# Autodesk Inventor assembly: манипулятор3
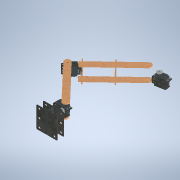
[picture p0: Inventor's stored thumbnail of the model, 180x180]
Saved by Autodesk Inventor 2020.1 (Build 241239000, 239)
## iProperties
Created: 2021-08-18
Part Number: манипулятор3
Document SubType Name: Assembly
Designer: User
Author: User
## Documents named in this file (8)
- D:\GitHub\avatar-kvantoriada\3D\манипулятор3.iam
- D:\GitHub\avatar-kvantoriada\3D\основа.ipt
- D:\GitHub\avatar-kvantoriada\3D\сборка серва 90.iam
- D:\GitHub\avatar-kvantoriada\3D\сборка серва 45_ЗЕРКАЛО2.iam
- D:\GitHub\avatar-kvantoriada\3D\Сборка1.iam
- D:\GitHub\avatar-kvantoriada\3D\уголок.ipt
- D:\GitHub\avatar-kvantoriada\3D\Сборка2.iam
- D:\GitHub\avatar-kvantoriada\3D\сборка серва 45.iam
## Components (9 placed, 7 different names)
1. основа:1 — Жесткий:1
2. основа:2 — Жесткий:1, Жесткий:2
3. сборка серва 90:1 [sub-assembly] — Жесткий:2, Жесткий:3
4. сборка серва 45_ЗЕРКАЛО2:1 [sub-assembly] — Жесткий:3, Жесткий:4
5. Сборка1:1 [sub-assembly] — Жесткий:4, Жесткий:5
6. сборка серва 90:2 [sub-assembly] — Жесткий:5, Жесткий:6
7. уголок:1 — Жесткий:6, Жесткий:7
8. Сборка2:1 [sub-assembly] — Жесткий:7
9. сборка серва 45:1 [sub-assembly]
## Relationships (7: WeldJoint 7)
- Жесткий:1 [WeldJoint]: основа:1 ↔ основа:2
- Жесткий:2 [WeldJoint]: основа:2 ↔ сборка серва 90:1
- Жесткий:3 [WeldJoint]: сборка серва 90:1 ↔ сборка серва 45_ЗЕРКАЛО2:1
- Жесткий:4 [WeldJoint]: сборка серва 45_ЗЕРКАЛО2:1 ↔ Сборка1:1
- Жесткий:5 [WeldJoint]: Сборка1:1 ↔ сборка серва 90:2
- Жесткий:6 [WeldJoint]: сборка серва 90:2 ↔ уголок:1
- Жесткий:7 [WeldJoint]: уголок:1 ↔ Сборка2:1
